# Autodesk Inventor assembly: A2017_T2_12
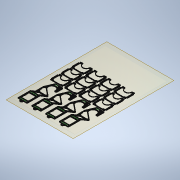
[picture p0: Inventor's stored thumbnail of the model, 180x180]
Saved by Autodesk Inventor 2020 (Build 240168000, 168)
## iProperties
Created: 2021-08-27
Part Number: A2017_T2_12
Document SubType Name: Assembly
Designer: Masato
Author: Masato
## Documents named in this file (4)
- D:\GitHub\inventor\SUSTAINA-OP\Cam\A2017_T2_12.iam
- D:\GitHub\inventor\SUSTAINA-OP\Cam\DisposableBoard.ipt
- D:\GitHub\inventor\SUSTAINA-OP\LowerBody\Ankle\Ankle_side_frame.ipt
- D:\GitHub\inventor\SUSTAINA-OP\LowerBody\Ankle\Ankle_back_frame.ipt
## Components (17 placed, 3 different names)
1. DisposableBoard:1 — メイト:2, メイト:1, フラッシュ:1, フラッシュ:2, メイト:5, フラッシュ:6, フラッシュ:8, メイト:6, フラッシュ:9
2. Ankle_back_frame:1 — メイト:6, フラッシュ:9, メイト:7
3. Ankle_back_frame:2
4. Ankle_back_frame:3
5. Ankle_back_frame:4
6. Ankle_back_frame:5
7. Ankle_back_frame:6
8. Ankle_back_frame:7
9. Ankle_back_frame:8
10. Ankle_back_frame:9
11. Ankle_back_frame:10
12. Ankle_back_frame:11
13. Ankle_back_frame:12
14. Ankle_side_frame:2 — メイト:5, フラッシュ:6, フラッシュ:8, メイト:7
15. Ankle_side_frame:3
16. Ankle_side_frame:4
17. Ankle_side_frame:5
## Component patterns: (1 elements), (12 elements, first: Ankle_back_frame:1), (4 elements, first: Ankle_side_frame:2)
## Relationships (10: Mate 5, Flush 5)
- メイト:2 [Mate]: DisposableBoard:1
- メイト:1 [Mate]: DisposableBoard:1
- フラッシュ:1 [Flush]: DisposableBoard:1
- フラッシュ:2 [Flush]: DisposableBoard:1
- メイト:5 [Mate]: DisposableBoard:1 ↔ Ankle_side_frame:2
- フラッシュ:6 [Flush] (4 mm): DisposableBoard:1 ↔ Ankle_side_frame:2
- フラッシュ:8 [Flush] (2 mm): DisposableBoard:1 ↔ Ankle_side_frame:2
- メイト:6 [Mate]: DisposableBoard:1 ↔ Ankle_back_frame:1
- フラッシュ:9 [Flush] (4 mm): DisposableBoard:1 ↔ Ankle_back_frame:1
- メイト:7 [Mate] (2.5 mm): Ankle_back_frame:1 ↔ Ankle_side_frame:2
